# Autodesk Inventor assembly: Turntable Ring Gear
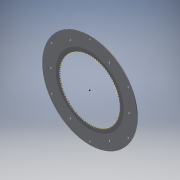
[picture p0: Inventor's stored thumbnail of the model, 180x180]
Saved by Autodesk Inventor 2016 (Build 200138000, 138)
## iProperties
Created: 2016-04-25
Part Number: Turntable Ring Gear
Document SubType Name: Assembly
Designer: rubenjm
Author: rubenjm
## Documents named in this file (3)
- C:\Users\rubenjm\Documents\To Transfer\2k16 Spring\RME\GGC\V3\Turntable Ring Gear.iam
- C:\Users\rubenjm\Documents\To Transfer\2k16 Spring\RME\GGC\V3\Turntable Outer Gear\Design Accelerator\Spur Gear22.ipt
- C:\Users\rubenjm\Documents\To Transfer\2k16 Spring\RME\GGC\V3\Ring Gear Outer.ipt
## Components (2 placed, 2 different names)
1. Spur Gear2:1 — Flush:1, Flush:2
2. Ring Gear Outer:1 — Flush:1, Flush:2
## Relationships (2: Flush 2)
- Flush:1: Spur Gear2:1 ↔ Ring Gear Outer:1
- Flush:2: Spur Gear2:1 ↔ Ring Gear Outer:1
